# Autodesk Inventor assembly: CasaGatoColgada
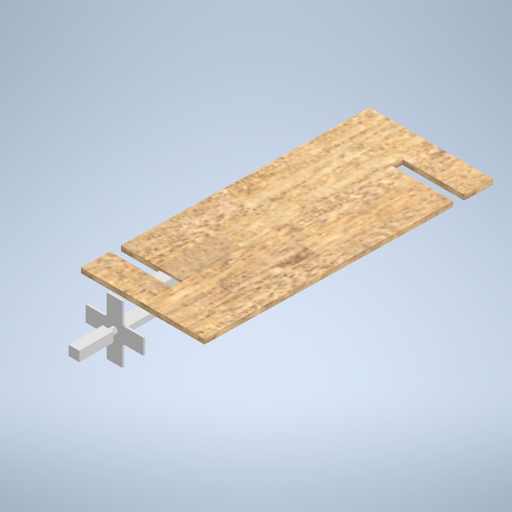
[picture p0: Inventor's stored thumbnail of the model, 512x512]
Saved by Autodesk Inventor 2023 (Build 270158000, 158)
## iProperties
Created: 2023-05-30
Part Number: CasaGatoColgada
Document SubType Name: Assembly
Designer: WIN10
Author: WIN10
## Documents named in this file (3)
- C:\Users\WIN10\DisenoDeProduccion\ModelosCeldaRobotica\CasaGatoColgada.iam
- C:\Users\WIN10\DisenoDeProduccion\ModelosCeldaRobotica\Gancho.ipt
- G:\Unidades compartidas\Amiguitos por siempre\APM 2023-1\Piezas\CGV1 Pieza Base.ipt
## Components (2 placed, 2 different names)
1. Gancho:1 — Coincidencia:1, Coincidencia:2, Coincidencia:3, Coincidencia:4, Coincidencia:5, Coincidencia:6
2. CGV1 Pieza Base:1 — Coincidencia:1, Coincidencia:2, Coincidencia:3
## Relationships (6: Mate 6)
- Coincidencia:1 [Mate]: Gancho:1 ↔ CGV1 Pieza Base:1
- Coincidencia:2 [Mate]: Gancho:1 ↔ CGV1 Pieza Base:1
- Coincidencia:3 [Mate]: Gancho:1 ↔ CGV1 Pieza Base:1
- Coincidencia:4 [Mate]: Gancho:1
- Coincidencia:5 [Mate]: Gancho:1
- Coincidencia:6 [Mate]: Gancho:1
